# Autodesk Inventor assembly: KimiFrontCover
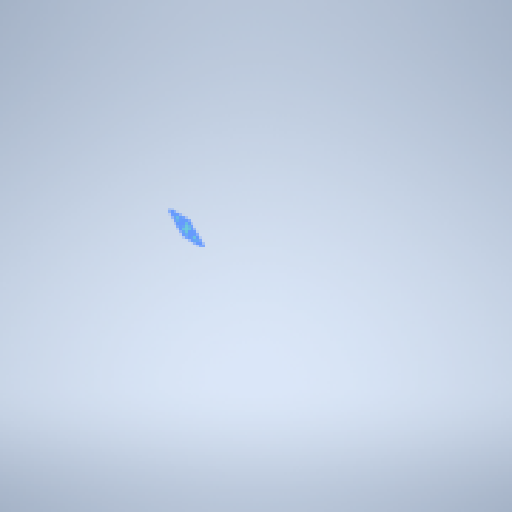
[picture p0: Inventor's stored thumbnail of the model, 512x512]
Saved by Autodesk Inventor 2025.1 (Build 291241000, 241)
## iProperties
Created: 2026-05-07
Part Number: KimiFrontCover
Document SubType Name: Assembly
Designer: User
Author: User
## Documents named in this file (3)
- D:\One Drive\OneDrive - Politeknik Sultan Salahuddin Abdul Aziz Shah\Documents\Inventor\RobosotPSA\KimiFrontCover.iam
- D:\One Drive\OneDrive - Politeknik Sultan Salahuddin Abdul Aziz Shah\Documents\Inventor\RobosotPSA\KimiBottomCover.ipt
- D:\One Drive\OneDrive - Politeknik Sultan Salahuddin Abdul Aziz Shah\Documents\Inventor\RobosotPSA\KimiRoofCover.ipt
## Components (2 placed, 2 different names)
1. KimiBottomCover:1 — Flush:1
2. KimiRoofCover:1 — Flush:1
## Relationships (1: Flush 1)
- Flush:1: KimiBottomCover:1 ↔ KimiRoofCover:1
